# Autodesk Inventor assembly: Проектирование сустава
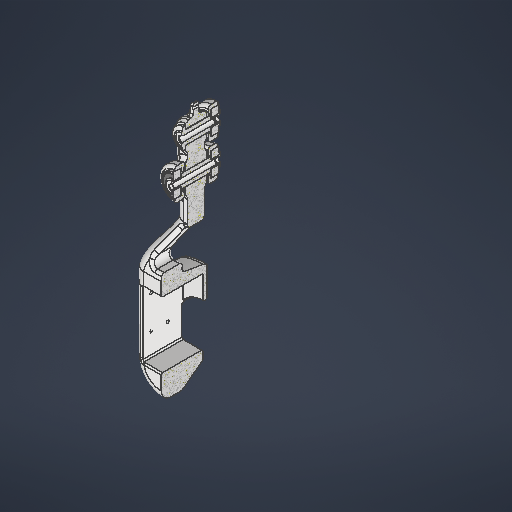
[picture p0: Inventor's stored thumbnail of the model, 512x512]
Saved by Autodesk Inventor 2025 (Build 290162010, 162A)
## iProperties
Created: 2024-12-06
Part Number: Проектирование сустава
Document SubType Name: Assembly
Designer: Edward_Higgins
Author: Edward_Higgins
## Documents named in this file (9)
- D:\Users\Edward_Higgins\Desktop\ZAVOD\Робот Сколково\Проектирование сустава.iam
- D:\Users\Edward_Higgins\Desktop\ZAVOD\Робот Сколково\Нога.ipt
- D:\Users\Edward_Higgins\Desktop\ZAVOD\Робот Сколково\Подшипник.ipt
- D:\Users\Edward_Higgins\Desktop\ZAVOD\Робот Сколково\Тяга передняя.ipt
- D:\Users\Edward_Higgins\Desktop\ZAVOD\Робот Сколково\Ось двусторонняя.ipt
- D:\Users\Edward_Higgins\Desktop\ZAVOD\Робот Сколково\Шайба.ipt
- D:\Users\Edward_Higgins\Desktop\ZAVOD\Робот Сколково\Стопорная шайба.ipt
- D:\Users\Edward_Higgins\Desktop\ZAVOD\Робот Сколково\Тяга задняя 2.ipt
- D:\Users\Edward_Higgins\Desktop\ZAVOD\Робот Сколково\Ось односторонняя.ipt
## Components (14 placed, 8 different names)
1. Нога:1 — Совмещение:1, Совмещение:2, Совмещение:3, Совмещение:9, Совмещение:10, Совмещение:15, Совмещение:16, Совмещение:23, Совмещение:28, Совмещение:29, Совмещение:32
2. Подшипник:1 — Совмещение:5, Совмещение:11, Совмещение:19
3. Тяга передняя:1 — Совмещение:3, Совмещение:5, Совмещение:7, Совмещение:9, Совмещение:21
4. Подшипник:2 — Совмещение:7, Совмещение:12, Совмещение:20, Совмещение:21
5. Ось двусторонняя:2 — Совмещение:10, Совмещение:11, Совмещение:12, Совмещение:13, Совмещение:14, Совмещение:17, Совмещение:18
6. Шайба:1 — Совмещение:13, Совмещение:16
7. Шайба:2 — Совмещение:14, Совмещение:15
8. Стопорная шайба:1 — Совмещение:18, Совмещение:19
9. Стопорная шайба:2 — Совмещение:17, Совмещение:20
10. Тяга задняя 2:1 — Совмещение:23, Совмещение:29, Совмещение:30, Совмещение:31
11. Подшипник:3 — Совмещение:25, Совмещение:26, Совмещение:30, Совмещение:31, Совмещение:33
12. Стопорная шайба:3 — Совмещение:25, Совмещение:26
13. Шайба:3 — Совмещение:28
14. Ось односторонняя:1 — Совмещение:32, Совмещение:33
## Relationships (27: Mate 27)
- Совмещение:1 [Mate]: Нога:1
- Совмещение:2 [Mate]: Нога:1
- Совмещение:3 [Mate]: Нога:1 ↔ Тяга передняя:1
- Совмещение:5 [Mate]: Подшипник:1 ↔ Тяга передняя:1
- Совмещение:7 [Mate]: Тяга передняя:1 ↔ Подшипник:2
- Совмещение:9 [Mate] (1 mm): Нога:1 ↔ Тяга передняя:1
- Совмещение:10 [Mate]: Нога:1 ↔ Ось двусторонняя:2
- Совмещение:11 [Mate]: Подшипник:1 ↔ Ось двусторонняя:2
- Совмещение:12 [Mate]: Подшипник:2 ↔ Ось двусторонняя:2
- Совмещение:13 [Mate]: Ось двусторонняя:2 ↔ Шайба:1
- Совмещение:14 [Mate]: Ось двусторонняя:2 ↔ Шайба:2
- Совмещение:15 [Mate]: Нога:1 ↔ Шайба:2
- Совмещение:16 [Mate]: Нога:1 ↔ Шайба:1
- Совмещение:17 [Mate]: Ось двусторонняя:2 ↔ Стопорная шайба:2
- Совмещение:18 [Mate]: Ось двусторонняя:2 ↔ Стопорная шайба:1
- Совмещение:19 [Mate]: Подшипник:1 ↔ Стопорная шайба:1
- Совмещение:20 [Mate]: Подшипник:2 ↔ Стопорная шайба:2
- Совмещение:21 [Mate] (0.25 mm): Тяга передняя:1 ↔ Подшипник:2
- Совмещение:23 [Mate] (1 mm): Нога:1 ↔ Тяга задняя 2:1
- Совмещение:25 [Mate]: Подшипник:3 ↔ Стопорная шайба:3
- Совмещение:26 [Mate]: Подшипник:3 ↔ Стопорная шайба:3
- Совмещение:28 [Mate]: Нога:1 ↔ Шайба:3
- Совмещение:29 [Mate]: Нога:1 ↔ Тяга задняя 2:1
- Совмещение:30 [Mate]: Тяга задняя 2:1 ↔ Подшипник:3
- Совмещение:31 [Mate]: Тяга задняя 2:1 ↔ Подшипник:3
- Совмещение:32 [Mate]: Нога:1 ↔ Ось односторонняя:1
- Совмещение:33 [Mate]: Подшипник:3 ↔ Ось односторонняя:1
